# Autodesk Inventor assembly: EnsamblajeDodecaedro_V3
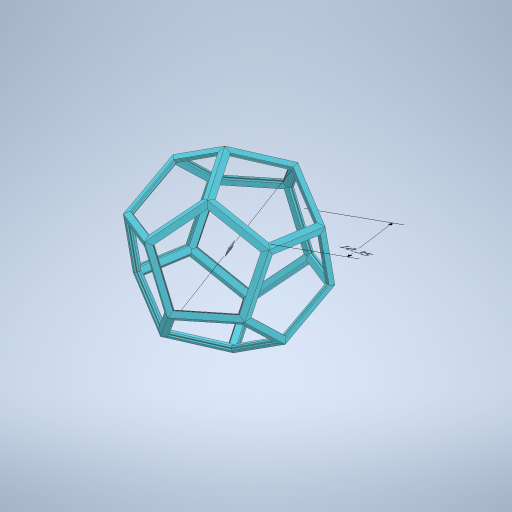
[picture p0: Inventor's stored thumbnail of the model, 512x512]
Saved by Autodesk Inventor 2024 (Build 280153000, 153)
## iProperties
Created: 2023-08-17
Part Number: EnsamblajeDodecaedro_V3
Document SubType Name: Assembly
Designer: sergi
Author: sergi
## Documents named in this file (2)
- C:\Users\sergi\OneDrive\Escritorio\Piso\Dodecaedro\EnsamblajeDodecaedro_V3.iam
- C:\Users\sergi\OneDrive\Escritorio\Piso\Dodecaedro\Perfil_V3.ipt
## Components (30 placed, 1 different names)
1. Perfil_V3:1 — Coincidencia:7, Coincidencia:8, Coincidencia:9, Coincidencia:57, Coincidencia:63
2. Perfil_V3:2 — Coincidencia:1, Coincidencia:2, Coincidencia:3, Coincidencia:5, Coincidencia:6, Coincidencia:43, Coincidencia:44, Coincidencia:45
3. Perfil_V3:3 — Coincidencia:1, Coincidencia:2, Coincidencia:3, Coincidencia:4, Coincidencia:7, Coincidencia:8, Coincidencia:9, Coincidencia:64, Coincidencia:65
4. Perfil_V3:4 — Coincidencia:4, Coincidencia:5, Coincidencia:6, Coincidencia:16, Coincidencia:17, Coincidencia:73
5. Perfil_V3:5 — Coincidencia:16, Coincidencia:17, Coincidencia:72
6. Perfil_V3:6 — Coincidencia:58, Coincidencia:59
7. Perfil_V3:7 — Coincidencia:29, Coincidencia:30, Coincidencia:31
8. Perfil_V3:8 — Coincidencia:30, Coincidencia:31
9. Perfil_V3:9 — Coincidencia:27, Coincidencia:28, Coincidencia:86
10. Perfil_V3:10 — Coincidencia:27, Coincidencia:28, Coincidencia:87, Coincidencia:88
11. Perfil_V3:11
12. Perfil_V3:12 — Coincidencia:29
13. Perfil_V3:13
14. Perfil_V3:14 — Coincidencia:43, Coincidencia:45
15. Perfil_V3:15 — Coincidencia:44
16. Perfil_V3:16
17. Perfil_V3:17
18. Perfil_V3:18 — Coincidencia:80, Coincidencia:81, Coincidencia:82, Coincidencia:83, Coincidencia:84, Coincidencia:85
19. Perfil_V3:19 — Coincidencia:60, Coincidencia:61
20. Perfil_V3:20 — Coincidencia:62
21. Perfil_V3:23 — Coincidencia:57, Coincidencia:58, Coincidencia:59, Coincidencia:60, Coincidencia:61, Coincidencia:62, Coincidencia:89
22. Perfil_V3:24 — Coincidencia:63, Coincidencia:64, Coincidencia:65, Coincidencia:66, Coincidencia:67, Coincidencia:68
23. Perfil_V3:25 — Coincidencia:66, Coincidencia:67, Coincidencia:68, Coincidencia:69, Coincidencia:70, Coincidencia:71
24. Perfil_V3:26 — Coincidencia:69, Coincidencia:70, Coincidencia:71
25. Perfil_V3:27 — Coincidencia:72, Coincidencia:73, Coincidencia:74, Coincidencia:75, Coincidencia:76, Coincidencia:77
26. Perfil_V3:28 — Coincidencia:74, Coincidencia:75, Coincidencia:76, Coincidencia:78, Coincidencia:79
27. Perfil_V3:29 — Coincidencia:77, Coincidencia:78, Coincidencia:79
28. Perfil_V3:30 — Coincidencia:80, Coincidencia:81, Coincidencia:82
29. Perfil_V3:31 — Coincidencia:83, Coincidencia:84, Coincidencia:85
30. Perfil_V3:32 — Coincidencia:86, Coincidencia:87, Coincidencia:88
## Relationships (84: Mate 84)
- Coincidencia:1 [Mate]: Perfil_V3:2 ↔ Perfil_V3:3
- Coincidencia:2 [Mate]: Perfil_V3:2 ↔ Perfil_V3:3
- Coincidencia:3 [Mate]: Perfil_V3:2 ↔ Perfil_V3:3
- Coincidencia:4 [Mate]: Perfil_V3:3 ↔ Perfil_V3:4
- Coincidencia:5 [Mate]: Perfil_V3:2 ↔ Perfil_V3:4
- Coincidencia:6 [Mate]: Perfil_V3:2 ↔ Perfil_V3:4
- Coincidencia:7 [Mate]: Perfil_V3:1 ↔ Perfil_V3:3
- Coincidencia:8 [Mate]: Perfil_V3:1 ↔ Perfil_V3:3
- Coincidencia:9 [Mate]: Perfil_V3:1 ↔ Perfil_V3:3
- [Mate]: Perfil_V3:5 ↔ Perfil_V3:6
- [Mate]: Perfil_V3:5 ↔ Perfil_V3:6
- [Mate]: Perfil_V3:5 ↔ Perfil_V3:6
- [Mate]: Perfil_V3:6 ↔ Perfil_V3:7
- [Mate]: Perfil_V3:5 ↔ Perfil_V3:7
- [Mate]: Perfil_V3:5 ↔ Perfil_V3:7
- Coincidencia:16 [Mate]: Perfil_V3:4 ↔ Perfil_V3:5
- Coincidencia:17 [Mate]: Perfil_V3:4 ↔ Perfil_V3:5
- [Mate]: Perfil_V3:9 ↔ Perfil_V3:10
- [Mate]: Perfil_V3:8 ↔ Perfil_V3:9
- [Mate]: Perfil_V3:8 ↔ Perfil_V3:9
- [Mate]: Perfil_V3:8 ↔ Perfil_V3:9
- [Mate]: Perfil_V3:11 ↔ Perfil_V3:12
- [Mate]: Perfil_V3:11 ↔ Perfil_V3:12
- [Mate]: Perfil_V3:11 ↔ Perfil_V3:12
- [Mate]: Perfil_V3:10 ↔ Perfil_V3:11
- [Mate]: Perfil_V3:10 ↔ Perfil_V3:11
- Coincidencia:27 [Mate]: Perfil_V3:9 ↔ Perfil_V3:10
- Coincidencia:28 [Mate]: Perfil_V3:9 ↔ Perfil_V3:10
- Coincidencia:29 [Mate]: Perfil_V3:7 ↔ Perfil_V3:12
- Coincidencia:30 [Mate]: Perfil_V3:7 ↔ Perfil_V3:8
- Coincidencia:31 [Mate]: Perfil_V3:7 ↔ Perfil_V3:8
- [Mate]: Perfil_V3:14 ↔ Perfil_V3:15
- [Mate]: Perfil_V3:13 ↔ Perfil_V3:14
- [Mate]: Perfil_V3:13 ↔ Perfil_V3:14
- [Mate]: Perfil_V3:13 ↔ Perfil_V3:14
- [Mate]: Perfil_V3:16 ↔ Perfil_V3:17
- [Mate]: Perfil_V3:16 ↔ Perfil_V3:17
- [Mate]: Perfil_V3:16 ↔ Perfil_V3:17
- [Mate]: Perfil_V3:15 ↔ Perfil_V3:16
- [Mate]: Perfil_V3:15 ↔ Perfil_V3:16
- [Mate]: Perfil_V3:14 ↔ Perfil_V3:15
- [Mate]: Perfil_V3:14 ↔ Perfil_V3:15
- Coincidencia:43 [Mate]: Perfil_V3:2 ↔ Perfil_V3:14
- Coincidencia:44 [Mate]: Perfil_V3:2 ↔ Perfil_V3:15
- Coincidencia:45 [Mate]: Perfil_V3:2 ↔ Perfil_V3:14
- [Mate]: Perfil_V3:19 ↔ Perfil_V3:20
- [Mate]: Perfil_V3:18 ↔ Perfil_V3:19
- [Mate]: Perfil_V3:18 ↔ Perfil_V3:19
- [Mate]: Perfil_V3:18 ↔ Perfil_V3:19
- [Mate]: Perfil_V3:19 ↔ Perfil_V3:20
- [Mate]: Perfil_V3:19 ↔ Perfil_V3:20
- Coincidencia:57 [Mate]: Perfil_V3:1 ↔ Perfil_V3:23
- Coincidencia:58 [Mate]: Perfil_V3:6 ↔ Perfil_V3:23
- Coincidencia:59 [Mate]: Perfil_V3:6 ↔ Perfil_V3:23
- Coincidencia:60 [Mate]: Perfil_V3:19 ↔ Perfil_V3:23
- Coincidencia:61 [Mate]: Perfil_V3:19 ↔ Perfil_V3:23
- Coincidencia:62 [Mate]: Perfil_V3:20 ↔ Perfil_V3:23
- Coincidencia:63 [Mate]: Perfil_V3:1 ↔ Perfil_V3:24
- Coincidencia:64 [Mate]: Perfil_V3:3 ↔ Perfil_V3:24
- Coincidencia:65 [Mate]: Perfil_V3:3 ↔ Perfil_V3:24
- Coincidencia:66 [Mate]: Perfil_V3:24 ↔ Perfil_V3:25
- Coincidencia:67 [Mate]: Perfil_V3:24 ↔ Perfil_V3:25
- Coincidencia:68 [Mate]: Perfil_V3:24 ↔ Perfil_V3:25
- Coincidencia:69 [Mate]: Perfil_V3:25 ↔ Perfil_V3:26
- Coincidencia:70 [Mate]: Perfil_V3:25 ↔ Perfil_V3:26
- Coincidencia:71 [Mate]: Perfil_V3:25 ↔ Perfil_V3:26
- Coincidencia:72 [Mate]: Perfil_V3:5 ↔ Perfil_V3:27
- Coincidencia:73 [Mate]: Perfil_V3:4 ↔ Perfil_V3:27
- Coincidencia:74 [Mate]: Perfil_V3:27 ↔ Perfil_V3:28
- Coincidencia:75 [Mate]: Perfil_V3:27 ↔ Perfil_V3:28
- Coincidencia:76 [Mate]: Perfil_V3:27 ↔ Perfil_V3:28
- Coincidencia:77 [Mate]: Perfil_V3:27 ↔ Perfil_V3:29
- Coincidencia:78 [Mate]: Perfil_V3:28 ↔ Perfil_V3:29
- Coincidencia:79 [Mate]: Perfil_V3:28 ↔ Perfil_V3:29
- Coincidencia:80 [Mate]: Perfil_V3:18 ↔ Perfil_V3:30
- Coincidencia:81 [Mate]: Perfil_V3:18 ↔ Perfil_V3:30
- Coincidencia:82 [Mate]: Perfil_V3:18 ↔ Perfil_V3:30
- Coincidencia:83 [Mate]: Perfil_V3:18 ↔ Perfil_V3:31
- Coincidencia:84 [Mate]: Perfil_V3:18 ↔ Perfil_V3:31
- Coincidencia:85 [Mate]: Perfil_V3:18 ↔ Perfil_V3:31
- Coincidencia:86 [Mate]: Perfil_V3:9 ↔ Perfil_V3:32
- Coincidencia:87 [Mate]: Perfil_V3:10 ↔ Perfil_V3:32
- Coincidencia:88 [Mate]: Perfil_V3:10 ↔ Perfil_V3:32
- Coincidencia:89 [Mate]: Perfil_V3:23
## Named parameters: d9_d2 = 0 mm, d10_d3 = 0 mm, d11_d4 = 0 mm, d12_d5 = 0 mm, d13_d0 = 0 mm, d14_d1 = 0 mm, d17_d15 = 0 mm, d18_d16 = 0 mm, d19_d3 = 0 mm, d20_d6 = 0 mm, d21_d7 = 0 mm, d22_d8 = 0 mm, d23_d9_d2 = 0 mm, d24_d13_d0 = 0 mm, d25_d14_d1 = 0 mm, d32_d17_d15 = 0 mm, d33_d18_d16 = 0 mm, d34_d19_d3 = 0 mm, d35_d20_d6 = 0 mm, d36_d21_d7 = 0 mm, d37_d22_d8 = 0 mm, d38_d23_d9_d2 = 0 mm, d39_d24_d13_d0 = 0 mm, d40_d25_d14_d1 = 0 mm, d41_d26 = 0 mm, d42_d27 = 0 mm, d48_d34_d19_d3 = 0 mm, d49_d35_d20_d6 = 0 mm, d50_d36_d21_d7 = 0 mm, d51_d37_d22_d8 = 0 mm, d55_d41_d26 = 0 mm, d56_d42_d27 = 0 mm
